# Autodesk Inventor assembly: patterndr
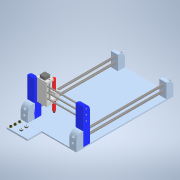
[picture p0: Inventor's stored thumbnail of the model, 180x180]
Saved by Autodesk Inventor 2022 (Build 260153070, 153G)
## iProperties
Created: 2021-07-07
Part Number: patterndr
Document SubType Name: Assembly
Designer: sachin
Author: sachin
## Documents named in this file (15)
- C:\Users\user\Downloads\patterndr (1).iam
- C:\Users\user\Downloads\board.ipt
- C:\Users\user\Downloads\rev rod (1).ipt
- C:\Users\user\Downloads\Part7.ipt
- C:\Users\user\Downloads\Part9.ipt
- C:\Users\user\Downloads\Part1 (2).ipt
- C:\Users\user\Downloads\Part3 (2).ipt
- C:\Users\user\Downloads\Part5 (2).ipt
- C:\Users\user\Downloads\Part4 (1).ipt
- C:\Users\user\Downloads\Part2113.ipt
- C:\Users\user\Downloads\rev pen.ipt
- C:\Users\user\Downloads\rev motor.ipt
- C:\Users\user\Downloads\Part121.ipt
- C:\Users\user\Downloads\buzzer.ipt
- C:\Users\user\Downloads\switch.ipt
## Components (24 placed, 14 different names)
1. board:1 — Rigid:1, Rotational:1, Rotational:2, Rotational:3, Flush:1, Mate:18, Mate:21, Flush:6
2. rev rod (1):1 — Rigid:1, Mate:1
3. rev rod (1):2 — Rotational:1, Mate:2
4. rev rod (1):3 — Rotational:2, Mate:3
5. rev rod (1):4 — Rotational:3, Mate:4
6. Part7:1 — Mate:1, Mate:2, Flush:1, Mate:5, Mate:8, Flush:3, Mate:10, Flush:4
7. Part7:2 — Mate:3, Mate:4, Mate:6, Flush:2, Mate:7, Mate:9, Mate:17, Mate:18
8. Part9:1 — Mate:5, Mate:6, Flush:2
9. Part9:2 — Mate:7, Mate:8, Flush:3, Mate:11
10. Part9:3 — Mate:9, Mate:10, Flush:4, Mate:12
11. Part1 (2):1 — Mate:11, Mate:12, Rigid:2, Rigid:3, Rigid:4, Mate:17, Mate:19, Flush:5, Mate:20, Rigid:7
12. Part3 (2):1 — Rigid:3
13. Part3 (2):2 — Rigid:2
14. Part5 (2):1 — Rigid:4
15. Part2113:1 — Mate:19, Flush:5, Rigid:5, Mate:20
16. Part4 (1):1 — Rigid:5, Rigid:6
17. rev pen:1 — Rigid:6
18. rev motor:1 — Rigid:7
19. Part121:1 — Mate:21, Flush:6, Mate:22, Mate:23, Mate:24, Mate:25, Mate:26
20. buzzer:1 — Mate:22
21. buzzer:2 — Mate:23
22. buzzer:3 — Mate:24
23. switch:2 — Mate:25
24. switch:3 — Mate:26
## Relationships (38: Mate 22, WeldJoint 7, Flush 6, RevoluteJoint 3)
- Rigid:1 [WeldJoint] (50.8 mm): board:1 ↔ rev rod (1):1
- Rotational:1 [RevoluteJoint] (50.8 mm): board:1 ↔ rev rod (1):2
- Rotational:2 [RevoluteJoint] (50.8 mm): board:1 ↔ rev rod (1):3
- Rotational:3 [RevoluteJoint] (50.8 mm): board:1 ↔ rev rod (1):4
- Mate:1: rev rod (1):1 ↔ Part7:1
- Mate:2: rev rod (1):2 ↔ Part7:1
- Flush:1: board:1 ↔ Part7:1
- Mate:3: rev rod (1):3 ↔ Part7:2
- Mate:4: rev rod (1):4 ↔ Part7:2
- Mate:5: Part7:1 ↔ Part9:1
- Mate:6: Part7:2 ↔ Part9:1
- Flush:2: Part7:2 ↔ Part9:1
- Mate:7: Part7:2 ↔ Part9:2
- Mate:8: Part7:1 ↔ Part9:2
- Flush:3: Part7:1 ↔ Part9:2
- Mate:9: Part7:2 ↔ Part9:3
- Mate:10: Part7:1 ↔ Part9:3
- Flush:4: Part7:1 ↔ Part9:3
- Mate:11: Part9:2 ↔ Part1 (2):1
- Mate:12: Part9:3 ↔ Part1 (2):1
- Rigid:2 [WeldJoint]: Part1 (2):1 ↔ Part3 (2):2
- Rigid:3 [WeldJoint]: Part1 (2):1 ↔ Part3 (2):1
- Rigid:4 [WeldJoint]: Part1 (2):1 ↔ Part5 (2):1
- Mate:17 (228.6 mm): Part7:2 ↔ Part1 (2):1
- Mate:18 (551.18 mm): board:1 ↔ Part7:2
- Mate:19: Part1 (2):1 ↔ Part2113:1
- Flush:5: Part1 (2):1 ↔ Part2113:1
- Rigid:5 [WeldJoint]: Part2113:1 ↔ Part4 (1):1
- Mate:20 (114.3 mm): Part1 (2):1 ↔ Part2113:1
- Rigid:6 [WeldJoint] (-25.4 mm): Part4 (1):1 ↔ rev pen:1
- Rigid:7 [WeldJoint]: Part1 (2):1 ↔ rev motor:1
- Mate:21: board:1 ↔ Part121:1
- Flush:6: board:1 ↔ Part121:1
- Mate:22: Part121:1 ↔ buzzer:1
- Mate:23: Part121:1 ↔ buzzer:2
- Mate:24: Part121:1 ↔ buzzer:3
- Mate:25: Part121:1 ↔ switch:2
- Mate:26: Part121:1 ↔ switch:3
